# Autodesk Inventor assembly: DroneDwiCakra
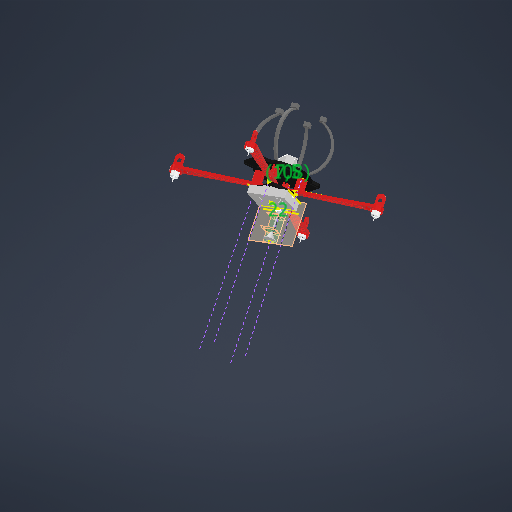
[picture p0: Inventor's stored thumbnail of the model, 512x512]
Saved by Autodesk Inventor 2026.1 (Build 301233000, 233)
## iProperties
Created: 2026-03-04
Part Number: DroneDwiCakra
Document SubType Name: Assembly
Designer: ayjuni03
Author: ayjuni03
## Documents named in this file (10)
- C:\Users\ayjuni03\Downloads\DroneDwiCakra.iam
- C:\Users\ayjuni03\Downloads\atasandrone.ipt
- C:\Users\ayjuni03\Downloads\sayapatas1.ipt
- C:\Users\ayjuni03\Downloads\dudukansayapdrone.ipt
- C:\Users\ayjuni03\Downloads\kakidrone.ipt
- C:\Users\ayjuni03\Downloads\brushless-motor-bldc_2212-6t-2200kv-1.snapshot.1\Motor_BLDC_2212,6T_2200KV\Motor_BLDC_2212,6T_2200KV\Motor_BLDC_2212,6T_2200KV.ipt
- C:\Users\ayjuni03\Downloads\gps  holder.ipt
- C:\Users\ayjuni03\Downloads\lid.ipt
- C:\Users\ayjuni03\Downloads\gps and fc holder ver 2.ipt
- C:\Users\ayjuni03\Downloads\batterycase.ipt
## Components (18 placed, 9 different names)
1. atasandrone:1 — Mate:1, Mate:2, Mate:3, Mate:4, Mate:5, Mate:6, Mate:7, Mate:8, Mate:9, Mate:14, Mate:15, Mate:16, Mate:45
2. sayapatas1:1 — Mate:1, Mate:2, Mate:10, Mate:17, Mate:20, Mate:39
3. sayapatas1:2 — Mate:7, Mate:8, Mate:14, Mate:23, Mate:40
4. sayapatas1:3 — Mate:5, Mate:6, Mate:15, Mate:21, Mate:22, Mate:38
5. sayapatas1:4 — Mate:3, Mate:4, Mate:16, Mate:18, Mate:19, Mate:35, Mate:36
6. dudukansayapdrone:1 — Mate:9, Mate:10, Mate:11, Mate:12, Mate:13, Mate:17, Mate:18, Mate:19, Mate:20, Mate:21, Mate:22, Mate:23, Mate:24, Mate:25, Mate:26, Mate:27, Mate:28, Mate:29, Mate:30, Mate:31, Mate:32, Mate:33, Mate:34, Mate:37
7. kakidrone:1 — Mate:11, Mate:12, Mate:24, Mate:37
8. kakidrone:2 — Mate:26, Mate:27, Mate:28, Mate:29, Mate:33
9. kakidrone:3 — Mate:30, Mate:31, Mate:32
10. kakidrone:4 — Mate:13, Mate:25, Mate:34
11. Motor_BLDC_2212,6T_2200KV:1 — Mate:35, Mate:36
12. Motor_BLDC_2212,6T_2200KV:2 — Mate:38
13. Motor_BLDC_2212,6T_2200KV:3 — Mate:40
14. Motor_BLDC_2212,6T_2200KV:4 — Mate:39
15. gps  holder:1 — Mate:41, Mate:42
16. lid:1 — Mate:43, Mate:44
17. gps and fc holder ver 2:1 — Mate:41, Mate:42, Mate:43, Mate:44, Mate:45
18. batterycase:1
## Relationships (45: Mate 45)
- Mate:1: atasandrone:1 ↔ sayapatas1:1
- Mate:2: atasandrone:1 ↔ sayapatas1:1
- Mate:3: atasandrone:1 ↔ sayapatas1:4
- Mate:4: atasandrone:1 ↔ sayapatas1:4
- Mate:5: atasandrone:1 ↔ sayapatas1:3
- Mate:6: atasandrone:1 ↔ sayapatas1:3
- Mate:7: atasandrone:1 ↔ sayapatas1:2
- Mate:8: atasandrone:1 ↔ sayapatas1:2
- Mate:9: atasandrone:1 ↔ dudukansayapdrone:1
- Mate:10: sayapatas1:1 ↔ dudukansayapdrone:1
- Mate:11: dudukansayapdrone:1 ↔ kakidrone:1
- Mate:12: dudukansayapdrone:1 ↔ kakidrone:1
- Mate:13: dudukansayapdrone:1 ↔ kakidrone:4
- Mate:14: atasandrone:1 ↔ sayapatas1:2
- Mate:15: atasandrone:1 ↔ sayapatas1:3
- Mate:16: atasandrone:1 ↔ sayapatas1:4
- Mate:17: sayapatas1:1 ↔ dudukansayapdrone:1
- Mate:18: sayapatas1:4 ↔ dudukansayapdrone:1
- Mate:19: sayapatas1:4 ↔ dudukansayapdrone:1
- Mate:20: sayapatas1:1 ↔ dudukansayapdrone:1
- Mate:21: sayapatas1:3 ↔ dudukansayapdrone:1
- Mate:22: sayapatas1:3 ↔ dudukansayapdrone:1
- Mate:23: sayapatas1:2 ↔ dudukansayapdrone:1
- Mate:24: dudukansayapdrone:1 ↔ kakidrone:1
- Mate:25: dudukansayapdrone:1 ↔ kakidrone:4
- Mate:26: dudukansayapdrone:1 ↔ kakidrone:2
- Mate:27: dudukansayapdrone:1 ↔ kakidrone:2
- Mate:28: dudukansayapdrone:1 ↔ kakidrone:2
- Mate:29: dudukansayapdrone:1 ↔ kakidrone:2
- Mate:30: dudukansayapdrone:1 ↔ kakidrone:3
- Mate:31: dudukansayapdrone:1 ↔ kakidrone:3
- Mate:32: dudukansayapdrone:1 ↔ kakidrone:3
- Mate:33: dudukansayapdrone:1 ↔ kakidrone:2
- Mate:34: dudukansayapdrone:1 ↔ kakidrone:4
- Mate:35: sayapatas1:4 ↔ Motor_BLDC_2212,6T_2200KV:1
- Mate:36: sayapatas1:4 ↔ Motor_BLDC_2212,6T_2200KV:1
- Mate:37: dudukansayapdrone:1 ↔ kakidrone:1
- Mate:38: sayapatas1:3 ↔ Motor_BLDC_2212,6T_2200KV:2
- Mate:39: sayapatas1:1 ↔ Motor_BLDC_2212,6T_2200KV:4
- Mate:40: sayapatas1:2 ↔ Motor_BLDC_2212,6T_2200KV:3
- Mate:41: gps  holder:1 ↔ gps and fc holder ver 2:1
- Mate:42: gps  holder:1 ↔ gps and fc holder ver 2:1
- Mate:43: lid:1 ↔ gps and fc holder ver 2:1
- Mate:44: lid:1 ↔ gps and fc holder ver 2:1
- Mate:45: atasandrone:1 ↔ gps and fc holder ver 2:1
## Named parameters: Finish1_Area = 3.14159, Finish2_Area = 303.541
note: some values were not read from the file. Shown as the stored number, unit unknown: "Finish1_Area", "Finish2_Area".
